# Autodesk Inventor assembly: box_layout_assm
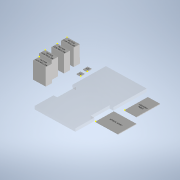
[picture p0: Inventor's stored thumbnail of the model, 180x180]
Saved by Autodesk Inventor 2020 (Build 240168000, 168)
## iProperties
Created: 2019-10-22
Part Number: box_layout_assm
Document SubType Name: Assembly
Designer: Connor
Author: Connor
## Documents named in this file (7)
- C:\Users\Connor\Desktop\KSU\2019 Fall\RMC\Electronics Box Layout\box_layout_assm.iam
- C:\Users\Connor\Desktop\KSU\2019 Fall\RMC\Electronics Box Layout\box_layout.ipt
- C:\Users\Connor\Desktop\KSU\2019 Fall\RMC\Electronics Box Layout\jetson_nano_sketch.ipt
- C:\Users\Connor\Desktop\KSU\2019 Fall\RMC\Electronics Box Layout\motor_controller_sketch.ipt
- C:\Users\Connor\Desktop\KSU\2019 Fall\RMC\Electronics Box Layout\mega_sketch.ipt
- C:\Users\Connor\Desktop\KSU\2019 Fall\RMC\Electronics Box Layout\24_12_step_down.ipt
- C:\Users\Connor\Desktop\KSU\2019 Fall\RMC\Electronics Box Layout\5V_step.ipt
## Components (9 placed, 6 different names)
1. jetson_nano_sketch:1 — Mate:4
2. box_layout:1 — Mate:1, Mate:2, Mate:4, Mate:23, Mate:24
3. mega_sketch:1 — Mate:15
4. motor_controller_sketch:1 — Mate:14
5. motor_controller_sketch:2 — Mate:13
6. motor_controller_sketch:3 — Mate:12
7. motor_controller_sketch:4 — Mate:11
8. 24_12_step_down:1 — Mate:23
9. 5V_step:1 — Mate:24
## Relationships (11: Mate 10, Flush 1)
- Mate:1: box_layout:1
- Mate:2: box_layout:1
- Mate:4: jetson_nano_sketch:1 ↔ box_layout:1
- Mate:11: motor_controller_sketch:4
- Mate:12: motor_controller_sketch:3
- Mate:13: motor_controller_sketch:2
- Mate:14: motor_controller_sketch:1
- Mate:15: mega_sketch:1
- Flush:1 (101.6 mm)
- Mate:23: box_layout:1 ↔ 24_12_step_down:1
- Mate:24: box_layout:1 ↔ 5V_step:1
